# Autodesk Inventor assembly: cum_holder_asembly
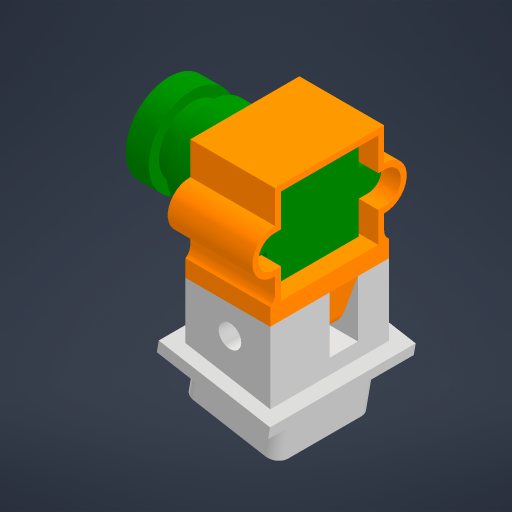
[picture p0: Inventor's stored thumbnail of the model, 512x512]
Saved by Autodesk Inventor 2024 (Build 280153000, 153)
## iProperties
Created: 2023-05-16
Part Number: cum_holder_asembly
Document SubType Name: Assembly
Designer: user
Author: user
## Documents named in this file (4)
- D:\Docs\Robot\3d\machine_body\cum_holders_mono\cum_holder_asembly.iam
- D:\Docs\Robot\3d\machine_body\cum_holder\cum_holder_up.ipt
- D:\Docs\Robot\3d\electronics\cum.ipt
- D:\Docs\Robot\3d\machine_body\cum_holders_mono\base_75.ipt
## Components (3 placed, 3 different names)
1. cum_holder_up:1 — Совмещение:3, Жесткий:1, Заподлицо:1
2. cum:1 — Совмещение:3, Жесткий:1
3. base_75:1 — Заподлицо:1
## Relationships (3: Mate 1, WeldJoint 1, Flush 1)
- Совмещение:3 [Mate]: cum_holder_up:1 ↔ cum:1
- Жесткий:1 [WeldJoint] (-3 mm): cum_holder_up:1 ↔ cum:1
- Заподлицо:1 [Flush]: cum_holder_up:1 ↔ base_75:1
